# Autodesk Inventor assembly: enix_assembly_v2
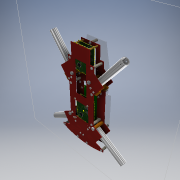
[picture p0: Inventor's stored thumbnail of the model, 180x180]
Saved by Autodesk Inventor 2016 (Build 200138000, 138)
## iProperties
Created: 2016-09-22
Part Number: enix_assembly_v2
Document SubType Name: Assembly
Designer: Jakub
Mass: 212.793 g
Surface Area: 2129.63 cm^2
Volume: 121.734 cm^3
Density: 1.74802 g/cm^3
Author: Jakub
## Documents named in this file (23)
- C:\Users\Jakub\Documents\DATA BANK\Projekty\Dron\Enix\V2\enix_assembly_v2.iam
- C:\Users\Jakub\Documents\DATA BANK\Projekty\Dron\Enix\V2\baseplate.ipt
- C:\Users\Jakub\Documents\DATA BANK\Projekty\Dron\Enix\V2\arm_grip.ipt
- C:\Users\Jakub\Documents\DATA BANK\Projekty\Dron\Enix\V2\arm_grip_mirror.ipt
- C:\Users\Jakub\Documents\DATA BANK\Projekty\Dron\Enix\V2\arm_front.ipt
- C:\Users\Jakub\Documents\DATA BANK\Projekty\Dron\Enix\V2\arm_back.ipt
- C:\Users\Jakub\Documents\DATA BANK\Projekty\Dron\Enix\V2\arm_lock.ipt
- C:\Users\Jakub\Documents\DATA BANK\Projekty\Dron\Enix\V2\dist25mm.ipt
- C:\Users\Jakub\Documents\Inventor\Content Center Files\R2016\en-US\AS 1427(04)\AS 1427 - M2 x 8(5) I.ipt
- C:\Users\Jakub\Documents\Inventor\Content Center Files\R2016\en-US\AS 1112 (2)\AS 1112 - M2  Type 5.ipt
- C:\Users\Jakub\Documents\DATA BANK\Projekty\Dron\Enix\V2\top_plate.ipt
- C:\Users\Jakub\Documents\Inventor\Content Center Files\R2016\en-US\UNI 6107\UNI 6107 - M4 x  30.ipt
- C:\Users\Jakub\Documents\Inventor\Content Center Files\R2016\en-US\ANSI B18.2.4.2M\ANSI B18.2.4.2M - M4x0,7 - 7.ipt
- C:\Users\Jakub\Documents\Inventor\Content Center Files\R2016\en-US\AS 1427(05)\AS 1427 - M3 x 5(5) II.ipt
- C:\Users\Jakub\Documents\DATA BANK\Projekty\Dron\Enix\V2\regulator.ipt
- C:\Users\Jakub\Documents\DATA BANK\Projekty\Dron\Enix\V2\dist10mmM2.ipt
- C:\Users\Jakub\Documents\Inventor\Content Center Files\R2016\en-US\ANSI B18.6.7M(01)\ANSI B18.6.7M - M2x0,4 x 5(5).ipt
- C:\Users\Jakub\Documents\DATA BANK\Projekty\Dron\Enix\V2\RASPBERRY PI 3.ipt
- C:\Users\Jakub\Documents\DATA BANK\Projekty\Dron\Enix\V2\dist5mmM2.ipt
- C:\Users\Jakub\Documents\DATA BANK\Projekty\Dron\Enix\V2\dist15mm.ipt
- C:\Users\Jakub\Documents\DATA BANK\Projekty\Dron\Enix\V2\cover.ipt
- C:\Users\Jakub\Documents\DATA BANK\Projekty\Dron\Enix\V2\kamera.ipt
- C:\Users\Jakub\Documents\DATA BANK\Projekty\Dron\Enix\V2\cam_holder.ipt
## Components (159 placed, 22 different names)
1. baseplate:1 — back_right_rot, front_right_rot, back_left_rot, front_left_rot, Mate:5, Mate:6, Mate:7, Mate:11, Mate:12, Mate:13, Mate:14, Mate:15, Mate:16, Mate:17, Mate:18, Mate:19, Mate:20, Mate:21, Mate:22, Mate:23, Mate:24, Mate:25, Mate:26, Mate:27, Mate:28, Mate:29, Mate:30, Mate:31, Mate:48, Mate:49, Mate:50, Mate:51, Mate:52, Mate:53, Mate:54, Mate:55, Mate:57, Mate:64, Mate:65, Mate:66, Mate:67, Mate:68, Mate:69, Mate:70, Mate:71, Mate:84, Mate:85, Mate:86, Mate:87, Mate:156, Mate:157, Mate:158, Mate:159, Mate:160, Mate:161, Mate:162, Mate:163, Mate:164, Mate:165, Mate:166, Mate:167, Mate:168, Mate:169, Mate:170, Mate:171, Mate:172, Mate:173, Mate:174, Mate:175, Mate:280, Mate:281, Mate:282, Mate:283, Mate:284, Mate:285, Mate:298, Mate:299, Mate:300, Mate:313, Mate:314, Mate:315, Mate:328, Mate:329
2. arm_grip:1 — back_right_rot, Mate:4, Flush:4, Angle:1, Mate:76
3. arm_grip:2 — front_right_rot, Mate:1, Flush:2, Mate:77
4. arm_grip_mirror:1 — back_left_rot, Mate:8, Flush:5, Angle:2, Mate:79
5. arm_grip_mirror:2 — front_left_rot, Mate:2, Flush:1, Mate:78
6. arm_front:1 — Mate:1, Flush:2
7. arm_front:2 — Mate:2, Flush:1
8. arm_back:1 — Mate:4, Flush:4, Angle:1
9. arm_back:2 — Mate:8, Flush:5, Angle:2
10. arm_lock:1 — Mate:5, Mate:6, Mate:7, Mate:32, Mate:33, Mate:38, Mate:39
11. arm_lock:2 — Mate:11, Mate:12, Mate:13, Mate:40, Mate:41, Mate:46, Mate:47
12. arm_lock:3 — Mate:14, Mate:15, Mate:16, Mate:42, Mate:43, Mate:44, Mate:45
13. arm_lock:4 — Mate:17, Mate:18, Mate:19, Mate:34, Mate:35, Mate:36, Mate:37
14. dist25mm:1 — Mate:20, Mate:23
15. dist25mm:2 — Mate:21, Mate:22
16. dist25mm:3 — Mate:27, Mate:28
17. dist25mm:4 — Mate:26, Mate:29
18. dist25mm:5 — Mate:25, Mate:30
19. dist25mm:6 — Mate:24, Mate:31, Mate:72, Mate:73
20. AS 1427 H - Metric M2 x 8:1 — Mate:32, Mate:38
21. AS 1427 H - Metric M2 x 8:2 — Mate:33, Mate:39, Mate:56
22. AS 1427 H - Metric M2 x 8:3 — Mate:34, Mate:36, Mate:63
23. AS 1427 H - Metric M2 x 8:4 — Mate:35, Mate:37, Mate:62
24. AS 1427 H - Metric M2 x 8:5 — Mate:42, Mate:44, Mate:60
25. AS 1427 H - Metric M2 x 8:6 — Mate:43, Mate:45, Mate:61
26. AS 1427 H - Metric M2 x 8:7 — Mate:41, Mate:46, Mate:58
27. AS 1427 H - Metric M2 x 8:8 — Mate:40, Mate:47, Mate:59
28. AS 1112 (2) - Metric M2  Type 5:1 — Mate:55, Mate:62
29. AS 1112 (2) - Metric M2  Type 5:2 — Mate:54, Mate:61
30. AS 1112 (2) - Metric M2  Type 5:3 — Mate:53, Mate:60
31. AS 1112 (2) - Metric M2  Type 5:4 — Mate:52, Mate:56
32. AS 1112 (2) - Metric M2  Type 5:5 — Mate:51, Mate:58
33. AS 1112 (2) - Metric M2  Type 5:6 — Mate:50, Mate:57
34. AS 1112 (2) - Metric M2  Type 5:7 — Mate:49, Mate:59
35. AS 1112 (2) - Metric M2  Type 5:8 — Mate:48, Mate:63
36. dist25mm:7 — Mate:68, Mate:69
37. dist25mm:8 — Mate:70, Mate:71, Mate:74
38. dist25mm:9 — Mate:66, Mate:67, Mate:75
39. dist25mm:10 — Mate:64, Mate:65
40. top_plate:1 — Mate:72, Mate:73, Mate:74, Mate:75, Mate:80, Mate:81, Mate:82, Mate:83, Mate:92, Mate:93, Mate:94, Mate:95, Mate:96, Mate:97, Mate:98, Mate:99, Mate:100, Mate:101, Mate:102, Mate:103, Mate:104, Mate:105, Mate:106, Mate:107, Mate:108, Mate:109, Mate:110, Mate:111, Mate:112, Mate:113, Mate:114, Mate:115, Mate:116, Mate:117, Mate:118, Mate:119, Mate:136, Mate:137, Mate:138, Mate:139, Mate:140, Mate:141, Mate:142, Mate:143, Mate:144, Mate:145, Mate:146, Mate:147, Mate:148, Mate:149, Mate:150, Mate:151, Mate:152, Mate:153, Mate:154, Mate:155, Mate:187, Mate:188, Mate:189, Mate:194, Mate:195, Mate:198, Mate:202, Mate:219, Mate:220, Mate:221, Mate:222, Mate:223, Mate:224, Mate:225, Mate:226, Mate:231, Mate:232, Mate:233, Mate:234, Mate:235, Mate:236, Mate:237, Mate:238, Mate:247, Mate:248, Mate:249, Mate:250, Mate:251, Mate:252, Mate:257, Mate:258, Mate:259, Mate:260, Mate:261, Mate:262, Mate:263, Mate:264, Mate:265, Mate:266
41. UNI 6107 M4 x  30:1 — Mate:76, Mate:81, Mate:89
42. UNI 6107 M4 x  30:2 — Mate:77, Mate:82, Mate:90
43. UNI 6107 M4 x  30:3 — Mate:78, Mate:83, Mate:91
44. UNI 6107 M4 x  30:4 — Mate:79, Mate:80, Mate:88
45. ANSI B18.2.4.2M M4x0,7:5 — Mate:87, Mate:91
46. ANSI B18.2.4.2M M4x0,7:6 — Mate:86, Mate:90
47. ANSI B18.2.4.2M M4x0,7:7 — Mate:85, Mate:88
48. ANSI B18.2.4.2M M4x0,7:8 — Mate:84, Mate:89
49. arm_lock:5 — Mate:92, Mate:93, Mate:94, Mate:132, Mate:133
50. arm_lock:6 — Mate:95, Mate:96, Mate:97, Mate:128, Mate:129
51. arm_lock:7 — Mate:98, Mate:99, Mate:100, Mate:120, Mate:121
52. arm_lock:8 — Mate:101, Mate:102, Mate:103, Mate:124, Mate:125
53. AS 1427 H - Metric M2 x 8:9 — Mate:108, Mate:118, Mate:131
54. AS 1427 H - Metric M2 x 8:10 — Mate:107, Mate:113, Mate:127
55. AS 1427 H - Metric M2 x 8:11 — Mate:109, Mate:119, Mate:130
56. AS 1427 H - Metric M2 x 8:12 — Mate:106, Mate:112, Mate:126
57. AS 1427 H - Metric M2 x 8:13 — Mate:110, Mate:117, Mate:135
58. AS 1427 H - Metric M2 x 8:14 — Mate:105, Mate:114, Mate:123
59. AS 1427 H - Metric M2 x 8:15 — Mate:111, Mate:116, Mate:134
60. AS 1427 H - Metric M2 x 8:16 — Mate:104, Mate:115, Mate:122
61. AS 1112 (2) - Metric M2  Type 5:9 — Mate:120, Mate:123
62. AS 1112 (2) - Metric M2  Type 5:10 — Mate:121, Mate:122
63. AS 1112 (2) - Metric M2  Type 5:11 — Mate:124, Mate:127
64. AS 1112 (2) - Metric M2  Type 5:12 — Mate:125, Mate:126
65. AS 1112 (2) - Metric M2  Type 5:13 — Mate:133, Mate:134
66. AS 1112 (2) - Metric M2  Type 5:14 — Mate:132, Mate:135
67. AS 1112 (2) - Metric M2  Type 5:15 — Mate:129, Mate:131
68. AS 1112 (2) - Metric M2  Type 5:16 — Mate:128, Mate:130
69. AS 1427 H - Metric M3 x 5:1 — Mate:137, Mate:145
70. AS 1427 H - Metric M3 x 5:2 — Mate:138, Mate:146
71. AS 1427 H - Metric M3 x 5:3 — Mate:154, Mate:155
72. AS 1427 H - Metric M3 x 5:4 — Mate:144, Mate:153
73. AS 1427 H - Metric M3 x 5:5 — Mate:143, Mate:151
74. AS 1427 H - Metric M3 x 5:6 — Mate:142, Mate:152
75. AS 1427 H - Metric M3 x 5:7 — Mate:141, Mate:149
76. AS 1427 H - Metric M3 x 5:8 — Mate:140, Mate:148
77. AS 1427 H - Metric M3 x 5:9 — Mate:139, Mate:147
78. AS 1427 H - Metric M3 x 5:10 — Mate:136, Mate:150
79. AS 1427 H - Metric M3 x 5:11 — Mate:165, Mate:166
80. AS 1427 H - Metric M3 x 5:12 — Mate:164, Mate:167
81. AS 1427 H - Metric M3 x 5:13 — Mate:163, Mate:168
82. AS 1427 H - Metric M3 x 5:14 — Mate:162, Mate:169
83. AS 1427 H - Metric M3 x 5:15 — Mate:161, Mate:170
84. AS 1427 H - Metric M3 x 5:16 — Mate:160, Mate:171
85. AS 1427 H - Metric M3 x 5:17 — Mate:159, Mate:172
86. AS 1427 H - Metric M3 x 5:18 — Mate:158, Mate:173
87. AS 1427 H - Metric M3 x 5:19 — Mate:157, Mate:175
88. AS 1427 H - Metric M3 x 5:20 — Mate:156, Mate:174
89. regulator:1 — Mate:176, Mate:177, Mate:178, Mate:179, Mate:190, Mate:191, Mate:192, Mate:193, Mate:199, Mate:200, Mate:201
90. regulator:2 — Mate:180, Mate:181, Mate:182, Mate:183, Mate:185
91. dist10mmM2:1 — Mate:177, Mate:179, Mate:182, Mate:184
92. dist10mmM2:2 — Mate:176, Mate:178, Mate:180, Mate:181, Mate:186
93. dist10mmM2:3 — Mate:183, Mate:184, Mate:189, Mate:197
94. dist10mmM2:4 — Mate:185, Mate:186, Mate:187, Mate:188, Mate:196
95. Cross Recessed Pan Head Machine Screw - Type IA - Metric M2x0,4 x 5:1 — Mate:191, Mate:192
96. Cross Recessed Pan Head Machine Screw - Type IA - Metric M2x0,4 x 5:2 — Mate:190, Mate:193
97. AS 1112 (2) - Metric M2  Type 5:17 — Mate:194, Mate:197
98. AS 1112 (2) - Metric M2  Type 5:18 — Mate:195, Mate:196
99. dist10mmM2:5 — Mate:198, Mate:203
100. dist10mmM2:6 — Mate:199
101. Cross Recessed Pan Head Machine Screw - Type IA - Metric M2x0,4 x 5:3 — Mate:200, Mate:201
102. AS 1112 (2) - Metric M2  Type 5:19 — Mate:202, Mate:203
103. RASPBERRY PI 3:1 — Mate:227, Mate:228, Mate:229, Mate:230, Mate:243, Mate:244, Mate:245, Mate:246
104. dist5mmM2:2 — Mate:221, Mate:225, Mate:228, Mate:240, Mate:253
105. dist5mmM2:3 — Mate:220, Mate:226, Mate:227, Mate:229, Mate:241, Mate:256
106. dist5mmM2:4 — Mate:219, Mate:223, Mate:230, Mate:242, Mate:255
107. dist5mmM2:5 — Mate:222, Mate:224, Mate:239, Mate:254
108. dist25mm:11 — Mate:233, Mate:234, Mate:269
109. dist25mm:12 — Mate:231, Mate:232, Mate:267, Mate:268
110. dist15mm:1 — Mate:235, Mate:237
111. dist15mm:2 — Mate:236, Mate:238
112. AS 1427 H - Metric M2 x 8:17 — Mate:239, Mate:243
113. AS 1427 H - Metric M2 x 8:18 — Mate:240, Mate:244
114. AS 1427 H - Metric M2 x 8:19 — Mate:241, Mate:245
115. AS 1427 H - Metric M2 x 8:20 — Mate:242, Mate:246
116. dist15mm:3 — Mate:247, Mate:248
117. AS 1112 (2) - Metric M2  Type 5:20 — Mate:249, Mate:253
118. AS 1112 (2) - Metric M2  Type 5:21 — Mate:250, Mate:254
119. AS 1112 (2) - Metric M2  Type 5:22 — Mate:251, Mate:256
120. AS 1112 (2) - Metric M2  Type 5:23 — Mate:252, Mate:255
121. AS 1427 H - Metric M3 x 5:21 — Mate:257, Mate:258
122. AS 1427 H - Metric M3 x 5:22 — Mate:259, Mate:260
123. AS 1427 H - Metric M3 x 5:23 — Mate:263, Mate:264
124. AS 1427 H - Metric M3 x 5:24 — Mate:265, Mate:266
125. AS 1427 H - Metric M3 x 5:25 — Mate:261, Mate:262
126. cover:1 — Mate:267, Mate:268, Mate:269, Mate:270, Mate:271, Mate:272, Mate:273, Mate:274, Mate:275, Mate:276, Mate:277, Mate:278, Mate:279
127. AS 1427 H - Metric M3 x 5:26 — Mate:274, Mate:275
128. AS 1427 H - Metric M3 x 5:27 — Mate:273, Mate:276
129. AS 1427 H - Metric M3 x 5:28 — Mate:272, Mate:277
130. AS 1427 H - Metric M3 x 5:29 — Mate:271, Mate:278
131. AS 1427 H - Metric M3 x 5:30 — Mate:270, Mate:279
132. dist5mmM2:6 — Mate:282, Mate:284, Mate:287, Mate:302
133. dist5mmM2:7 — Mate:281, Mate:283, Mate:286, Mate:288, Mate:301
134. dist5mmM2:8 — Mate:280, Mate:285, Mate:303
135. regulator:3 — Mate:286, Mate:287, Mate:288, Mate:289, Mate:290, Mate:291, Mate:292, Mate:293, Mate:294
136. regulator:4 — Mate:295, Mate:296, Mate:297, Mate:304, Mate:305, Mate:306, Mate:307, Mate:308, Mate:309
137. dist10mmM2:7 — Mate:291, Mate:293, Mate:295, Mate:296
138. dist10mmM2:8 — Mate:290, Mate:294, Mate:297
139. dist10mmM2:9 — Mate:289, Mate:292
140. AS 1112 (2) - Metric M2  Type 5:24 — Mate:298, Mate:302
141. AS 1112 (2) - Metric M2  Type 5:25 — Mate:300, Mate:303
142. AS 1112 (2) - Metric M2  Type 5:26 — Mate:299, Mate:301
143. AS 1427 H - Metric M2 x 8:21 — Mate:308, Mate:309
144. AS 1427 H - Metric M2 x 8:22 — Mate:306, Mate:307
145. AS 1427 H - Metric M2 x 8:23 — Mate:304, Mate:305
146. kamera:1 — Mate:310, Mate:311, Mate:312, Mate:320, Mate:321, Mate:322, Mate:323, Mate:324, Mate:325, Mate:326, Mate:327
147. cam_holder:1 — Mate:310, Mate:311, Mate:312, Mate:313, Mate:314, Mate:315, Mate:316, Mate:317, Mate:318, Mate:319, Mate:332, Mate:333, Mate:334, Mate:335
148. AS 1427 H - Metric M2 x 8:24 — Mate:317, Mate:319, Mate:330
149. AS 1427 H - Metric M2 x 8:25 — Mate:326, Mate:327, Mate:339
150. AS 1427 H - Metric M2 x 8:26 — Mate:324, Mate:325, Mate:338
151. AS 1427 H - Metric M2 x 8:27 — Mate:320, Mate:321, Mate:336
152. AS 1427 H - Metric M2 x 8:28 — Mate:316, Mate:318, Mate:331
153. AS 1427 H - Metric M2 x 8:29 — Mate:322, Mate:323, Mate:337
154. AS 1112 (2) - Metric M2  Type 5:27 — Mate:329, Mate:330
155. AS 1112 (2) - Metric M2  Type 5:28 — Mate:328, Mate:331
156. AS 1112 (2) - Metric M2  Type 5:29 — Mate:332, Mate:339
157. AS 1112 (2) - Metric M2  Type 5:30 — Mate:333, Mate:338
158. AS 1112 (2) - Metric M2  Type 5:31 — Mate:334, Mate:337
159. AS 1112 (2) - Metric M2  Type 5:32 — Mate:335, Mate:336
## Relationships (331: Mate 321, RevoluteJoint 4, Flush 4, Angle 2)
- back_right_rot [RevoluteJoint]: baseplate:1 ↔ arm_grip:1
- front_right_rot [RevoluteJoint]: baseplate:1 ↔ arm_grip:2
- back_left_rot [RevoluteJoint]: baseplate:1 ↔ arm_grip_mirror:1
- front_left_rot [RevoluteJoint]: baseplate:1 ↔ arm_grip_mirror:2
- Mate:1: arm_grip:2 ↔ arm_front:1
- Mate:2: arm_grip_mirror:2 ↔ arm_front:2
- Flush:1: arm_grip_mirror:2 ↔ arm_front:2
- Flush:2: arm_grip:2 ↔ arm_front:1
- Mate:4: arm_grip:1 ↔ arm_back:1
- Flush:4: arm_grip:1 ↔ arm_back:1
- Mate:5: baseplate:1 ↔ arm_lock:1
- Mate:6: baseplate:1 ↔ arm_lock:1
- Mate:7: baseplate:1 ↔ arm_lock:1
- Angle:1 (0 deg): arm_grip:1 ↔ arm_back:1
- Mate:8: arm_grip_mirror:1 ↔ arm_back:2
- Flush:5: arm_grip_mirror:1 ↔ arm_back:2
- Angle:2 (0 deg): arm_grip_mirror:1 ↔ arm_back:2
- Mate:11: baseplate:1 ↔ arm_lock:2
- Mate:12: baseplate:1 ↔ arm_lock:2
- Mate:13: baseplate:1 ↔ arm_lock:2
- Mate:14: baseplate:1 ↔ arm_lock:3
- Mate:15: baseplate:1 ↔ arm_lock:3
- Mate:16: baseplate:1 ↔ arm_lock:3
- Mate:17: baseplate:1 ↔ arm_lock:4
- Mate:18: baseplate:1 ↔ arm_lock:4
- Mate:19: baseplate:1 ↔ arm_lock:4
- Mate:20: baseplate:1 ↔ dist25mm:1
- Mate:21: baseplate:1 ↔ dist25mm:2
- Mate:22: baseplate:1 ↔ dist25mm:2
- Mate:23: baseplate:1 ↔ dist25mm:1
- Mate:24: baseplate:1 ↔ dist25mm:6
- Mate:25: baseplate:1 ↔ dist25mm:5
- Mate:26: baseplate:1 ↔ dist25mm:4
- Mate:27: baseplate:1 ↔ dist25mm:3
- Mate:28: baseplate:1 ↔ dist25mm:3
- Mate:29: baseplate:1 ↔ dist25mm:4
- Mate:30: baseplate:1 ↔ dist25mm:5
- Mate:31: baseplate:1 ↔ dist25mm:6
- Mate:32: arm_lock:1 ↔ AS 1427 H - Metric M2 x 8:1
- Mate:33: arm_lock:1 ↔ AS 1427 H - Metric M2 x 8:2
- Mate:34: arm_lock:4 ↔ AS 1427 H - Metric M2 x 8:3
- Mate:35: arm_lock:4 ↔ AS 1427 H - Metric M2 x 8:4
- Mate:36: arm_lock:4 ↔ AS 1427 H - Metric M2 x 8:3
- Mate:37: arm_lock:4 ↔ AS 1427 H - Metric M2 x 8:4
- Mate:38: arm_lock:1 ↔ AS 1427 H - Metric M2 x 8:1
- Mate:39: arm_lock:1 ↔ AS 1427 H - Metric M2 x 8:2
- Mate:40: arm_lock:2 ↔ AS 1427 H - Metric M2 x 8:8
- Mate:41: arm_lock:2 ↔ AS 1427 H - Metric M2 x 8:7
- Mate:42: arm_lock:3 ↔ AS 1427 H - Metric M2 x 8:5
- Mate:43: arm_lock:3 ↔ AS 1427 H - Metric M2 x 8:6
- Mate:44: arm_lock:3 ↔ AS 1427 H - Metric M2 x 8:5
- Mate:45: arm_lock:3 ↔ AS 1427 H - Metric M2 x 8:6
- Mate:46: arm_lock:2 ↔ AS 1427 H - Metric M2 x 8:7
- Mate:47: arm_lock:2 ↔ AS 1427 H - Metric M2 x 8:8
- Mate:48: baseplate:1 ↔ AS 1112 (2) - Metric M2  Type 5:8
- Mate:49: baseplate:1 ↔ AS 1112 (2) - Metric M2  Type 5:7
- Mate:50: baseplate:1 ↔ AS 1112 (2) - Metric M2  Type 5:6
- Mate:51: baseplate:1 ↔ AS 1112 (2) - Metric M2  Type 5:5
- Mate:52: baseplate:1 ↔ AS 1112 (2) - Metric M2  Type 5:4
- Mate:53: baseplate:1 ↔ AS 1112 (2) - Metric M2  Type 5:3
- Mate:54: baseplate:1 ↔ AS 1112 (2) - Metric M2  Type 5:2
- Mate:55: baseplate:1 ↔ AS 1112 (2) - Metric M2  Type 5:1
- Mate:56: AS 1427 H - Metric M2 x 8:2 ↔ AS 1112 (2) - Metric M2  Type 5:4
- Mate:57: baseplate:1 ↔ AS 1112 (2) - Metric M2  Type 5:6
- Mate:58: AS 1427 H - Metric M2 x 8:7 ↔ AS 1112 (2) - Metric M2  Type 5:5
- Mate:59: AS 1427 H - Metric M2 x 8:8 ↔ AS 1112 (2) - Metric M2  Type 5:7
- Mate:60: AS 1427 H - Metric M2 x 8:5 ↔ AS 1112 (2) - Metric M2  Type 5:3
- Mate:61: AS 1427 H - Metric M2 x 8:6 ↔ AS 1112 (2) - Metric M2  Type 5:2
- Mate:62: AS 1427 H - Metric M2 x 8:4 ↔ AS 1112 (2) - Metric M2  Type 5:1
- Mate:63: AS 1427 H - Metric M2 x 8:3 ↔ AS 1112 (2) - Metric M2  Type 5:8
- Mate:64: baseplate:1 ↔ dist25mm:10
- Mate:65: baseplate:1 ↔ dist25mm:10
- Mate:66: baseplate:1 ↔ dist25mm:9
- Mate:67: baseplate:1 ↔ dist25mm:9
- Mate:68: baseplate:1 ↔ dist25mm:7
- Mate:69: baseplate:1 ↔ dist25mm:7
- Mate:70: baseplate:1 ↔ dist25mm:8
- Mate:71: baseplate:1 ↔ dist25mm:8
- Mate:72: dist25mm:6 ↔ top_plate:1
- Mate:73: dist25mm:6 ↔ top_plate:1
- Mate:74: dist25mm:8 ↔ top_plate:1
- Mate:75: dist25mm:9 ↔ top_plate:1
- Mate:76: arm_grip:1 ↔ UNI 6107 M4 x  30:1
- Mate:77: arm_grip:2 ↔ UNI 6107 M4 x  30:2
- Mate:78: arm_grip_mirror:2 ↔ UNI 6107 M4 x  30:3
- Mate:79: arm_grip_mirror:1 ↔ UNI 6107 M4 x  30:4
- Mate:80: top_plate:1 ↔ UNI 6107 M4 x  30:4
- Mate:81: top_plate:1 ↔ UNI 6107 M4 x  30:1
- Mate:82: top_plate:1 ↔ UNI 6107 M4 x  30:2
- Mate:83: top_plate:1 ↔ UNI 6107 M4 x  30:3
- Mate:84: baseplate:1 ↔ ANSI B18.2.4.2M M4x0,7:8
- Mate:85: baseplate:1 ↔ ANSI B18.2.4.2M M4x0,7:7
- Mate:86: baseplate:1 ↔ ANSI B18.2.4.2M M4x0,7:6
- Mate:87: baseplate:1 ↔ ANSI B18.2.4.2M M4x0,7:5
- Mate:88: UNI 6107 M4 x  30:4 ↔ ANSI B18.2.4.2M M4x0,7:7
- Mate:89: UNI 6107 M4 x  30:1 ↔ ANSI B18.2.4.2M M4x0,7:8
- Mate:90: UNI 6107 M4 x  30:2 ↔ ANSI B18.2.4.2M M4x0,7:6
- Mate:91: UNI 6107 M4 x  30:3 ↔ ANSI B18.2.4.2M M4x0,7:5
- Mate:92: top_plate:1 ↔ arm_lock:5
- Mate:93: top_plate:1 ↔ arm_lock:5
- Mate:94: top_plate:1 ↔ arm_lock:5
- Mate:95: top_plate:1 ↔ arm_lock:6
- Mate:96: top_plate:1 ↔ arm_lock:6
- Mate:97: top_plate:1 ↔ arm_lock:6
- Mate:98: top_plate:1 ↔ arm_lock:7
- Mate:99: top_plate:1 ↔ arm_lock:7
- Mate:100: top_plate:1 ↔ arm_lock:7
- Mate:101: top_plate:1 ↔ arm_lock:8
- Mate:102: top_plate:1 ↔ arm_lock:8
- Mate:103: top_plate:1 ↔ arm_lock:8
- Mate:104: top_plate:1 ↔ AS 1427 H - Metric M2 x 8:16
- Mate:105: top_plate:1 ↔ AS 1427 H - Metric M2 x 8:14
- Mate:106: top_plate:1 ↔ AS 1427 H - Metric M2 x 8:12
- Mate:107: top_plate:1 ↔ AS 1427 H - Metric M2 x 8:10
- Mate:108: top_plate:1 ↔ AS 1427 H - Metric M2 x 8:9
- Mate:109: top_plate:1 ↔ AS 1427 H - Metric M2 x 8:11
- Mate:110: top_plate:1 ↔ AS 1427 H - Metric M2 x 8:13
- Mate:111: top_plate:1 ↔ AS 1427 H - Metric M2 x 8:15
- Mate:112: top_plate:1 ↔ AS 1427 H - Metric M2 x 8:12
- Mate:113: top_plate:1 ↔ AS 1427 H - Metric M2 x 8:10
- Mate:114: top_plate:1 ↔ AS 1427 H - Metric M2 x 8:14
- Mate:115: top_plate:1 ↔ AS 1427 H - Metric M2 x 8:16
- Mate:116: top_plate:1 ↔ AS 1427 H - Metric M2 x 8:15
- Mate:117: top_plate:1 ↔ AS 1427 H - Metric M2 x 8:13
- Mate:118: top_plate:1 ↔ AS 1427 H - Metric M2 x 8:9
- Mate:119: top_plate:1 ↔ AS 1427 H - Metric M2 x 8:11
- Mate:120: arm_lock:7 ↔ AS 1112 (2) - Metric M2  Type 5:9
- Mate:121: arm_lock:7 ↔ AS 1112 (2) - Metric M2  Type 5:10
- Mate:122: AS 1427 H - Metric M2 x 8:16 ↔ AS 1112 (2) - Metric M2  Type 5:10
- Mate:123: AS 1427 H - Metric M2 x 8:14 ↔ AS 1112 (2) - Metric M2  Type 5:9
- Mate:124: arm_lock:8 ↔ AS 1112 (2) - Metric M2  Type 5:11
- Mate:125: arm_lock:8 ↔ AS 1112 (2) - Metric M2  Type 5:12
- Mate:126: AS 1427 H - Metric M2 x 8:12 ↔ AS 1112 (2) - Metric M2  Type 5:12
- Mate:127: AS 1427 H - Metric M2 x 8:10 ↔ AS 1112 (2) - Metric M2  Type 5:11
- Mate:128: arm_lock:6 ↔ AS 1112 (2) - Metric M2  Type 5:16
- Mate:129: arm_lock:6 ↔ AS 1112 (2) - Metric M2  Type 5:15
- Mate:130: AS 1427 H - Metric M2 x 8:11 ↔ AS 1112 (2) - Metric M2  Type 5:16
- Mate:131: AS 1427 H - Metric M2 x 8:9 ↔ AS 1112 (2) - Metric M2  Type 5:15
- Mate:132: arm_lock:5 ↔ AS 1112 (2) - Metric M2  Type 5:14
- Mate:133: arm_lock:5 ↔ AS 1112 (2) - Metric M2  Type 5:13
- Mate:134: AS 1427 H - Metric M2 x 8:15 ↔ AS 1112 (2) - Metric M2  Type 5:13
- Mate:135: AS 1427 H - Metric M2 x 8:13 ↔ AS 1112 (2) - Metric M2  Type 5:14
- Mate:136: top_plate:1 ↔ AS 1427 H - Metric M3 x 5:10
- Mate:137: top_plate:1 ↔ AS 1427 H - Metric M3 x 5:1
- Mate:138: top_plate:1 ↔ AS 1427 H - Metric M3 x 5:2
- Mate:139: top_plate:1 ↔ AS 1427 H - Metric M3 x 5:9
- Mate:140: top_plate:1 ↔ AS 1427 H - Metric M3 x 5:8
- Mate:141: top_plate:1 ↔ AS 1427 H - Metric M3 x 5:7
- Mate:142: top_plate:1 ↔ AS 1427 H - Metric M3 x 5:6
- Mate:143: top_plate:1 ↔ AS 1427 H - Metric M3 x 5:5
- Mate:144: top_plate:1 ↔ AS 1427 H - Metric M3 x 5:4
- Mate:145: top_plate:1 ↔ AS 1427 H - Metric M3 x 5:1
- Mate:146: top_plate:1 ↔ AS 1427 H - Metric M3 x 5:2
- Mate:147: top_plate:1 ↔ AS 1427 H - Metric M3 x 5:9
- Mate:148: top_plate:1 ↔ AS 1427 H - Metric M3 x 5:8
- Mate:149: top_plate:1 ↔ AS 1427 H - Metric M3 x 5:7
- Mate:150: top_plate:1 ↔ AS 1427 H - Metric M3 x 5:10
- Mate:151: top_plate:1 ↔ AS 1427 H - Metric M3 x 5:5
- Mate:152: top_plate:1 ↔ AS 1427 H - Metric M3 x 5:6
- Mate:153: top_plate:1 ↔ AS 1427 H - Metric M3 x 5:4
- Mate:154: top_plate:1 ↔ AS 1427 H - Metric M3 x 5:3
- Mate:155: top_plate:1 ↔ AS 1427 H - Metric M3 x 5:3
- Mate:156: baseplate:1 ↔ AS 1427 H - Metric M3 x 5:20
- Mate:157: baseplate:1 ↔ AS 1427 H - Metric M3 x 5:19
- Mate:158: baseplate:1 ↔ AS 1427 H - Metric M3 x 5:18
- Mate:159: baseplate:1 ↔ AS 1427 H - Metric M3 x 5:17
- Mate:160: baseplate:1 ↔ AS 1427 H - Metric M3 x 5:16
- Mate:161: baseplate:1 ↔ AS 1427 H - Metric M3 x 5:15
- Mate:162: baseplate:1 ↔ AS 1427 H - Metric M3 x 5:14
- Mate:163: baseplate:1 ↔ AS 1427 H - Metric M3 x 5:13
- Mate:164: baseplate:1 ↔ AS 1427 H - Metric M3 x 5:12
- Mate:165: baseplate:1 ↔ AS 1427 H - Metric M3 x 5:11
- Mate:166: baseplate:1 ↔ AS 1427 H - Metric M3 x 5:11
- Mate:167: baseplate:1 ↔ AS 1427 H - Metric M3 x 5:12
- Mate:168: baseplate:1 ↔ AS 1427 H - Metric M3 x 5:13
- Mate:169: baseplate:1 ↔ AS 1427 H - Metric M3 x 5:14
- Mate:170: baseplate:1 ↔ AS 1427 H - Metric M3 x 5:15
- Mate:171: baseplate:1 ↔ AS 1427 H - Metric M3 x 5:16
- Mate:172: baseplate:1 ↔ AS 1427 H - Metric M3 x 5:17
- Mate:173: baseplate:1 ↔ AS 1427 H - Metric M3 x 5:18
- Mate:174: baseplate:1 ↔ AS 1427 H - Metric M3 x 5:20
- Mate:175: baseplate:1 ↔ AS 1427 H - Metric M3 x 5:19
- Mate:176: regulator:1 ↔ dist10mmM2:2
- Mate:177: regulator:1 ↔ dist10mmM2:1
- Mate:178: regulator:1 ↔ dist10mmM2:2
- Mate:179: regulator:1 ↔ dist10mmM2:1
- Mate:180: regulator:2 ↔ dist10mmM2:2
- Mate:181: regulator:2 ↔ dist10mmM2:2
- Mate:182: regulator:2 ↔ dist10mmM2:1
- Mate:183: regulator:2 ↔ dist10mmM2:3
- Mate:184: dist10mmM2:1 ↔ dist10mmM2:3
- Mate:185: regulator:2 ↔ dist10mmM2:4
- Mate:186: dist10mmM2:2 ↔ dist10mmM2:4
- Mate:187: top_plate:1 ↔ dist10mmM2:4
- Mate:188: top_plate:1 ↔ dist10mmM2:4
- Mate:189: top_plate:1 ↔ dist10mmM2:3
- Mate:190: regulator:1 ↔ Cross Recessed Pan Head Machine Screw - Type IA - Metric M2x0,4 x 5:2
- Mate:191: regulator:1 ↔ Cross Recessed Pan Head Machine Screw - Type IA - Metric M2x0,4 x 5:1
- Mate:192: regulator:1 ↔ Cross Recessed Pan Head Machine Screw - Type IA - Metric M2x0,4 x 5:1
- Mate:193: regulator:1 ↔ Cross Recessed Pan Head Machine Screw - Type IA - Metric M2x0,4 x 5:2
- Mate:194: top_plate:1 ↔ AS 1112 (2) - Metric M2  Type 5:17
- Mate:195: top_plate:1 ↔ AS 1112 (2) - Metric M2  Type 5:18
- Mate:196: dist10mmM2:4 ↔ AS 1112 (2) - Metric M2  Type 5:18
- Mate:197: dist10mmM2:3 ↔ AS 1112 (2) - Metric M2  Type 5:17
- Mate:198: top_plate:1 ↔ dist10mmM2:5
- Mate:199: regulator:1 ↔ dist10mmM2:6
- Mate:200: regulator:1 ↔ Cross Recessed Pan Head Machine Screw - Type IA - Metric M2x0,4 x 5:3
- Mate:201: regulator:1 ↔ Cross Recessed Pan Head Machine Screw - Type IA - Metric M2x0,4 x 5:3
- Mate:202: top_plate:1 ↔ AS 1112 (2) - Metric M2  Type 5:19
- Mate:203: dist10mmM2:5 ↔ AS 1112 (2) - Metric M2  Type 5:19
- Mate:219: top_plate:1 ↔ dist5mmM2:4
- Mate:220: top_plate:1 ↔ dist5mmM2:3
- Mate:221: top_plate:1 ↔ dist5mmM2:2
- Mate:222: top_plate:1 ↔ dist5mmM2:5
- Mate:223: top_plate:1 ↔ dist5mmM2:4
- Mate:224: top_plate:1 ↔ dist5mmM2:5
- Mate:225: top_plate:1 ↔ dist5mmM2:2
- Mate:226: top_plate:1 ↔ dist5mmM2:3
- Mate:227: RASPBERRY PI 3:1 ↔ dist5mmM2:3
- Mate:228: RASPBERRY PI 3:1 ↔ dist5mmM2:2
- Mate:229: RASPBERRY PI 3:1 ↔ dist5mmM2:3
- Mate:230: RASPBERRY PI 3:1 ↔ dist5mmM2:4
- Mate:231: top_plate:1 ↔ dist25mm:12
- Mate:232: top_plate:1 ↔ dist25mm:12
- Mate:233: top_plate:1 ↔ dist25mm:11
- Mate:234: top_plate:1 ↔ dist25mm:11
- Mate:235: top_plate:1 ↔ dist15mm:1
- Mate:236: top_plate:1 ↔ dist15mm:2
- Mate:237: top_plate:1 ↔ dist15mm:1
- Mate:238: top_plate:1 ↔ dist15mm:2
- Mate:239: dist5mmM2:5 ↔ AS 1427 H - Metric M2 x 8:17
- Mate:240: dist5mmM2:2 ↔ AS 1427 H - Metric M2 x 8:18
- Mate:241: dist5mmM2:3 ↔ AS 1427 H - Metric M2 x 8:19
- Mate:242: dist5mmM2:4 ↔ AS 1427 H - Metric M2 x 8:20
- Mate:243: RASPBERRY PI 3:1 ↔ AS 1427 H - Metric M2 x 8:17
- Mate:244: RASPBERRY PI 3:1 ↔ AS 1427 H - Metric M2 x 8:18
- Mate:245: RASPBERRY PI 3:1 ↔ AS 1427 H - Metric M2 x 8:19
- Mate:246: RASPBERRY PI 3:1 ↔ AS 1427 H - Metric M2 x 8:20
- Mate:247: top_plate:1 ↔ dist15mm:3
- Mate:248: top_plate:1 ↔ dist15mm:3
- Mate:249: top_plate:1 ↔ AS 1112 (2) - Metric M2  Type 5:20
- Mate:250: top_plate:1 ↔ AS 1112 (2) - Metric M2  Type 5:21
- Mate:251: top_plate:1 ↔ AS 1112 (2) - Metric M2  Type 5:22
- Mate:252: top_plate:1 ↔ AS 1112 (2) - Metric M2  Type 5:23
- Mate:253: dist5mmM2:2 ↔ AS 1112 (2) - Metric M2  Type 5:20
- Mate:254: dist5mmM2:5 ↔ AS 1112 (2) - Metric M2  Type 5:21
- Mate:255: dist5mmM2:4 ↔ AS 1112 (2) - Metric M2  Type 5:23
- Mate:256: dist5mmM2:3 ↔ AS 1112 (2) - Metric M2  Type 5:22
- Mate:257: top_plate:1 ↔ AS 1427 H - Metric M3 x 5:21
- Mate:258: top_plate:1 ↔ AS 1427 H - Metric M3 x 5:21
- Mate:259: top_plate:1 ↔ AS 1427 H - Metric M3 x 5:22
- Mate:260: top_plate:1 ↔ AS 1427 H - Metric M3 x 5:22
- Mate:261: top_plate:1 ↔ AS 1427 H - Metric M3 x 5:25
- Mate:262: top_plate:1 ↔ AS 1427 H - Metric M3 x 5:25
- Mate:263: top_plate:1 ↔ AS 1427 H - Metric M3 x 5:23
- Mate:264: top_plate:1 ↔ AS 1427 H - Metric M3 x 5:23
- Mate:265: top_plate:1 ↔ AS 1427 H - Metric M3 x 5:24
- Mate:266: top_plate:1 ↔ AS 1427 H - Metric M3 x 5:24
- Mate:267: dist25mm:12 ↔ cover:1
- Mate:268: dist25mm:12 ↔ cover:1
- Mate:269: dist25mm:11 ↔ cover:1
- Mate:270: cover:1 ↔ AS 1427 H - Metric M3 x 5:30
- Mate:271: cover:1 ↔ AS 1427 H - Metric M3 x 5:29
- Mate:272: cover:1 ↔ AS 1427 H - Metric M3 x 5:28
- Mate:273: cover:1 ↔ AS 1427 H - Metric M3 x 5:27
- Mate:274: cover:1 ↔ AS 1427 H - Metric M3 x 5:26
- Mate:275: cover:1 ↔ AS 1427 H - Metric M3 x 5:26
- Mate:276: cover:1 ↔ AS 1427 H - Metric M3 x 5:27
- Mate:277: cover:1 ↔ AS 1427 H - Metric M3 x 5:28
- Mate:278: cover:1 ↔ AS 1427 H - Metric M3 x 5:29
- Mate:279: cover:1 ↔ AS 1427 H - Metric M3 x 5:30
- Mate:280: baseplate:1 ↔ dist5mmM2:8
- Mate:281: baseplate:1 ↔ dist5mmM2:7
- Mate:282: baseplate:1 ↔ dist5mmM2:6
- Mate:283: baseplate:1 ↔ dist5mmM2:7
- Mate:284: baseplate:1 ↔ dist5mmM2:6
- Mate:285: baseplate:1 ↔ dist5mmM2:8
- Mate:286: dist5mmM2:7 ↔ regulator:3
- Mate:287: dist5mmM2:6 ↔ regulator:3
- Mate:288: dist5mmM2:7 ↔ regulator:3
- Mate:289: regulator:3 ↔ dist10mmM2:9
- Mate:290: regulator:3 ↔ dist10mmM2:8
- Mate:291: regulator:3 ↔ dist10mmM2:7
- Mate:292: regulator:3 ↔ dist10mmM2:9
- Mate:293: regulator:3 ↔ dist10mmM2:7
- Mate:294: regulator:3 ↔ dist10mmM2:8
- Mate:295: regulator:4 ↔ dist10mmM2:7
- Mate:296: regulator:4 ↔ dist10mmM2:7
- Mate:297: regulator:4 ↔ dist10mmM2:8
- Mate:298: baseplate:1 ↔ AS 1112 (2) - Metric M2  Type 5:24
- Mate:299: baseplate:1 ↔ AS 1112 (2) - Metric M2  Type 5:26
- Mate:300: baseplate:1 ↔ AS 1112 (2) - Metric M2  Type 5:25
- Mate:301: dist5mmM2:7 ↔ AS 1112 (2) - Metric M2  Type 5:26
- Mate:302: dist5mmM2:6 ↔ AS 1112 (2) - Metric M2  Type 5:24
- Mate:303: dist5mmM2:8 ↔ AS 1112 (2) - Metric M2  Type 5:25
- Mate:304: regulator:4 ↔ AS 1427 H - Metric M2 x 8:23
- Mate:305: regulator:4 ↔ AS 1427 H - Metric M2 x 8:23
- Mate:306: regulator:4 ↔ AS 1427 H - Metric M2 x 8:22
- Mate:307: regulator:4 ↔ AS 1427 H - Metric M2 x 8:22
- Mate:308: regulator:4 ↔ AS 1427 H - Metric M2 x 8:21
- Mate:309: regulator:4 ↔ AS 1427 H - Metric M2 x 8:21
- Mate:310: kamera:1 ↔ cam_holder:1
- Mate:311: kamera:1 ↔ cam_holder:1
- Mate:312: kamera:1 ↔ cam_holder:1
- Mate:313: baseplate:1 ↔ cam_holder:1
- Mate:314: baseplate:1 ↔ cam_holder:1
- Mate:315: baseplate:1 ↔ cam_holder:1
- Mate:316: cam_holder:1 ↔ AS 1427 H - Metric M2 x 8:28
- Mate:317: cam_holder:1 ↔ AS 1427 H - Metric M2 x 8:24
- Mate:318: cam_holder:1 ↔ AS 1427 H - Metric M2 x 8:28
- Mate:319: cam_holder:1 ↔ AS 1427 H - Metric M2 x 8:24
- Mate:320: kamera:1 ↔ AS 1427 H - Metric M2 x 8:27
- Mate:321: kamera:1 ↔ AS 1427 H - Metric M2 x 8:27
- Mate:322: kamera:1 ↔ AS 1427 H - Metric M2 x 8:29
- Mate:323: kamera:1 ↔ AS 1427 H - Metric M2 x 8:29
- Mate:324: kamera:1 ↔ AS 1427 H - Metric M2 x 8:26
- Mate:325: kamera:1 ↔ AS 1427 H - Metric M2 x 8:26
- Mate:326: kamera:1 ↔ AS 1427 H - Metric M2 x 8:25
- Mate:327: kamera:1 ↔ AS 1427 H - Metric M2 x 8:25
- Mate:328: baseplate:1 ↔ AS 1112 (2) - Metric M2  Type 5:28
- Mate:329: baseplate:1 ↔ AS 1112 (2) - Metric M2  Type 5:27
- Mate:330: AS 1427 H - Metric M2 x 8:24 ↔ AS 1112 (2) - Metric M2  Type 5:27
- Mate:331: AS 1427 H - Metric M2 x 8:28 ↔ AS 1112 (2) - Metric M2  Type 5:28
- Mate:332: cam_holder:1 ↔ AS 1112 (2) - Metric M2  Type 5:29
- Mate:333: cam_holder:1 ↔ AS 1112 (2) - Metric M2  Type 5:30
- Mate:334: cam_holder:1 ↔ AS 1112 (2) - Metric M2  Type 5:31
- Mate:335: cam_holder:1 ↔ AS 1112 (2) - Metric M2  Type 5:32
- Mate:336: AS 1427 H - Metric M2 x 8:27 ↔ AS 1112 (2) - Metric M2  Type 5:32
- Mate:337: AS 1427 H - Metric M2 x 8:29 ↔ AS 1112 (2) - Metric M2  Type 5:31
- Mate:338: AS 1427 H - Metric M2 x 8:26 ↔ AS 1112 (2) - Metric M2  Type 5:30
- Mate:339: AS 1427 H - Metric M2 x 8:25 ↔ AS 1112 (2) - Metric M2  Type 5:29
## Named parameters: sa_0 = -13.8611, sa_1 = 0, sa_2 = 999.904, sa_3 = -5.52663, sa_4 = 0, sa_5 = 999.985, sa_6 = 0, sa_7 = -500, sa_8 = -0
note: some values were not read from the file. Shown as the stored number, unit unknown: "sa_0", "sa_1", "sa_2", "sa_3", "sa_4", "sa_5", "sa_6", "sa_7", "sa_8".
